# Autodesk Inventor assembly: Zmotionassembly(right)
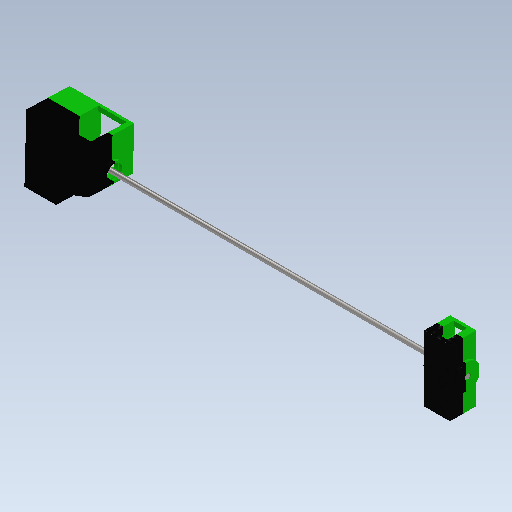
[picture p0: Inventor's stored thumbnail of the model, 512x512]
Saved by Autodesk Inventor 2020.4 (Build 244396000, 396)
## iProperties
Created: 2021-03-29
Part Number: Zmotionassembly(right)
Document SubType Name: Assembly
Designer: AOB
Mass: 241.781 g
Surface Area: 690.311 cm^2
Volume: 133.74 cm^3
Density: 1.80785 g/cm^3
Author: AOB
## Documents named in this file (4)
- C:\Users\marti\Documents\Inventor\ProjectBoron\Boron Ultima\Zmotionassembly(right).iam
- C:\Users\marti\Documents\Inventor\ProjectBoron\Boron Ultima\Z-powertrain(right).iam
- C:\Users\marti\Documents\Inventor\ProjectBoron\Boron Ultima\bottom idler housing(right).iam
- C:\Users\marti\Documents\Inventor\ProjectBoron\Boron Ultima\zmotorblock(right).iam
## Components (3 placed, 3 different names)
1. Z-powertrain(right):1 [sub-assembly] — Flush:1, Mate:2, Flush:2, Mate:3
2. bottom idler housing(right):1 [sub-assembly] — Flush:1, Mate:2
3. zmotorblock(right):1 [sub-assembly] — Flush:2, Mate:3
## Relationships (4: Flush 2, Mate 2)
- Flush:1: Z-powertrain(right):1 ↔ bottom idler housing(right):1
- Mate:2: Z-powertrain(right):1 ↔ bottom idler housing(right):1
- Flush:2: Z-powertrain(right):1 ↔ zmotorblock(right):1
- Mate:3: Z-powertrain(right):1 ↔ zmotorblock(right):1
